# Autodesk Inventor assembly: Shield
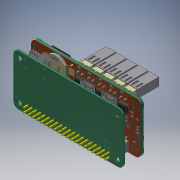
[picture p0: Inventor's stored thumbnail of the model, 180x180]
Saved by Autodesk Inventor 2017 (Build 210142000, 142)
## iProperties
Created: 2017-09-23
Part Number: Shield
Document SubType Name: Assembly
Designer: P. Baesso
Author: P. Baesso
## Documents named in this file (6)
- C:\Rymapt\ethoscope_hardware\Shield\Shield.iam
- C:\Rymapt\ethoscope_hardware\PiZero\RapberryPiZero.iam
- C:\Rymapt\ethoscope_hardware\Shield\Files\User Library-CR1225.iam
- C:\Rymapt\ethoscope_hardware\Shield\Files\PCB_R2D2.iam
- C:\Rymapt\ethoscope_hardware\Shield\Files\PCB_MTLW-120-07-G-D-250.iam
- C:\Rymapt\ethoscope_hardware\Shield\Files\022012021.ipt
## Components (9 placed, 5 different names)
1. RapberryPiZero:1 [sub-assembly] — Flush:2, Flush:3, Mate:1, Mate:2, Mate:3, Angle:1
2. User Library-CR1225:1 [sub-assembly] — Flush:4, Tangent:1, Tangent:2
3. PCB_R2D2:1 [sub-assembly] — Flush:2, Flush:3, Flush:4, Tangent:1, Tangent:2, Mate:7, Flush:6, Flush:7, Mate:8
4. PCB_MTLW-120-07-G-D-250:1 [sub-assembly] — Mate:1, Mate:2, Mate:3, Angle:1, Mate:8
5. 022012021:1 — Mate:7, Flush:6, Flush:7
6. 022012021:2
7. 022012021:3
8. 022012021:4
9. 022012021:5
## Component patterns: CableConnector (5 elements)
## Relationships (13: Flush 5, Mate 5, Tangent 2, Angle 1)
- Flush:2: RapberryPiZero:1 ↔ PCB_R2D2:1
- Flush:3: RapberryPiZero:1 ↔ PCB_R2D2:1
- Flush:4 (0.1 mm): User Library-CR1225:1 ↔ PCB_R2D2:1
- Tangent:1 (0.1 mm): User Library-CR1225:1 ↔ PCB_R2D2:1
- Tangent:2 (0.15 mm): User Library-CR1225:1 ↔ PCB_R2D2:1
- Mate:1: RapberryPiZero:1 ↔ PCB_MTLW-120-07-G-D-250:1
- Mate:2 (-0.32 mm): RapberryPiZero:1 ↔ PCB_MTLW-120-07-G-D-250:1
- Mate:3 (-0.32 mm): RapberryPiZero:1 ↔ PCB_MTLW-120-07-G-D-250:1
- Angle:1 (0 deg): RapberryPiZero:1 ↔ PCB_MTLW-120-07-G-D-250:1
- Mate:7: PCB_R2D2:1 ↔ 022012021:1
- Flush:6 (-0.28 mm): PCB_R2D2:1 ↔ 022012021:1
- Flush:7 (-0.3 mm): PCB_R2D2:1 ↔ 022012021:1
- Mate:8 (1 mm): PCB_R2D2:1 ↔ PCB_MTLW-120-07-G-D-250:1
